# Autodesk Inventor assembly: Delrin and Aluminum Spool
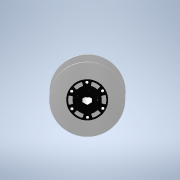
[picture p0: Inventor's stored thumbnail of the model, 180x180]
Saved by Autodesk Inventor 2020 (Build 240168000, 168)
## iProperties
Created: 2020-02-04
Part Number: Delrin and Aluminum Spool
Document SubType Name: Assembly
Designer: JimAndVal
Author: JimAndVal
## Documents named in this file (4)
- D:\Users\JimAndVal\Documents\JIM\IronRiders\2020 Robot-1\Climber\Delrin and Aluminum Spool.iam
- D:\Users\JimAndVal\Documents\JIM\IronRiders\2020 Robot-1\Climber\Spool Hub.ipt
- D:\Users\JimAndVal\Documents\JIM\IronRiders\2020 Robot-1\Climber\Spool Plate.ipt
- D:\Users\JimAndVal\Documents\JIM\IronRiders\2020 Robot-1\Climber\1_2_Hex_Bore_Aluminum_VersaHub_217-2592.ipt
## Components (6 placed, 3 different names)
1. Spool Hub:1 — Mate:2, Mate:7, Mate:8, Mate:13
2. Spool Hub:2 — Mate:3, Mate:8, Mate:9, Mate:12
3. Spool Plate:1 — Mate:1, Mate:6, Mate:7, Mate:14
4. Spool Plate:2 — Mate:4, Mate:9, Mate:10, Mate:11
5. 1_2_Hex_Bore_Aluminum_VersaHub_217-2592:1 — Mate:1, Mate:2, Mate:3, Mate:4, Mate:5, Mate:6, Mate:15
6. 1_2_Hex_Bore_Aluminum_VersaHub_217-2592:2 — Mate:5, Mate:10, Flush:1
## Relationships (16: Mate 15, Flush 1)
- Mate:1: Spool Plate:1 ↔ 1_2_Hex_Bore_Aluminum_VersaHub_217-2592:1
- Mate:2: Spool Hub:1 ↔ 1_2_Hex_Bore_Aluminum_VersaHub_217-2592:1
- Mate:3: Spool Hub:2 ↔ 1_2_Hex_Bore_Aluminum_VersaHub_217-2592:1
- Mate:4: Spool Plate:2 ↔ 1_2_Hex_Bore_Aluminum_VersaHub_217-2592:1
- Mate:5: 1_2_Hex_Bore_Aluminum_VersaHub_217-2592:1 ↔ 1_2_Hex_Bore_Aluminum_VersaHub_217-2592:2
- Mate:6: Spool Plate:1 ↔ 1_2_Hex_Bore_Aluminum_VersaHub_217-2592:1
- Mate:7: Spool Hub:1 ↔ Spool Plate:1
- Mate:8: Spool Hub:1 ↔ Spool Hub:2
- Mate:9: Spool Hub:2 ↔ Spool Plate:2
- Mate:10: Spool Plate:2 ↔ 1_2_Hex_Bore_Aluminum_VersaHub_217-2592:2
- Flush:1: 1_2_Hex_Bore_Aluminum_VersaHub_217-2592:2
- Mate:11: Spool Plate:2
- Mate:12: Spool Hub:2
- Mate:13: Spool Hub:1
- Mate:14: Spool Plate:1
- Mate:15: 1_2_Hex_Bore_Aluminum_VersaHub_217-2592:1
